# Autodesk Inventor assembly: gears
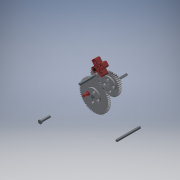
[picture p0: Inventor's stored thumbnail of the model, 180x180]
Saved by Autodesk Inventor 2019 (Build 230136000, 136)
## iProperties
Created: 2019-01-24
Part Number: gears
Document SubType Name: Assembly
Designer: Varga Daniel
Author: Varga Daniel
## Documents named in this file (8)
- C:\!_Dani\!_cloud\OneDrive\!_munka\Revolution\RevvyDemoKit\Structural parts\Demo parts\Gears\gears.iam
- C:\!_Dani\!_cloud\OneDrive\!_munka\Revolution\RevvyDemoKit\Structural parts\Connetor Pins\cp1x1.ipt
- C:\!_Dani\!_cloud\OneDrive\!_munka\Revolution\RevvyDemoKit\Structural parts\Axle Connectors\Axle connector 3x3 cross.ipt
- C:\!_Dani\!_cloud\OneDrive\!_munka\Revolution\RevvyDemoKit\Structural parts\Demo parts\Gears\gear40.iam
- C:\!_Dani\!_cloud\OneDrive\!_munka\Revolution\RevvyDemoKit\Structural parts\Axles\Axle 2.ipt
- C:\!_Dani\!_cloud\OneDrive\!_munka\Revolution\RevvyDemoKit\Structural parts\Demo parts\Gears\gear60.iam
- C:\!_Dani\!_cloud\OneDrive\!_munka\Revolution\RevvyDemoKit\Structural parts\Axles\Axle 5s.ipt
- C:\!_Dani\!_cloud\OneDrive\!_munka\Revolution\RevvyDemoKit\Structural parts\Demo parts\Gears\gear20.iam
## Components (12 placed, 7 different names)
1. cp1x1:1 — Mate:3, Mate:4
2. gear40:1 [sub-assembly] — Mate:12, Mate:13, Flush:1, Mate:16, Mate:18, Mate:19, Mate:20
3. Axle connector 3x3 cross:2 — Mate:3, Mate:4
4. gear60:1 [sub-assembly] — Mate:8, Mate:9, Mate:10, Mate:11, Flush:2, Mate:17, Angle:1, Mate:18
5. Axle 2:3
6. Axle 2:4 — Mate:8, Mate:9, Angle:1
7. cp1x1:2 — Mate:10, Mate:11
8. Axle 5s:1
9. Axle 5s:2 — Mate:12, Mate:13
10. gear20:1 [sub-assembly] — Mate:14, Mate:15, Flush:1, Mate:16, Flush:2, Mate:17
11. Axle 5s:3 — Mate:14, Mate:15
12. gear20:2 [sub-assembly] — Mate:19, Mate:20
## Relationships (18: Mate 15, Flush 2, Angle 1)
- Mate:3: cp1x1:1 ↔ Axle connector 3x3 cross:2
- Mate:4: cp1x1:1 ↔ Axle connector 3x3 cross:2
- Mate:8: gear60:1 ↔ Axle 2:4
- Mate:9: gear60:1 ↔ Axle 2:4
- Mate:10: gear60:1 ↔ cp1x1:2
- Mate:11: gear60:1 ↔ cp1x1:2
- Mate:12: gear40:1 ↔ Axle 5s:2
- Mate:13: gear40:1 ↔ Axle 5s:2
- Mate:14: gear20:1 ↔ Axle 5s:3
- Mate:15: gear20:1 ↔ Axle 5s:3
- Flush:1: gear40:1 ↔ gear20:1
- Mate:16 (30 mm): gear40:1 ↔ gear20:1
- Flush:2: gear60:1 ↔ gear20:1
- Mate:17 (40 mm): gear60:1 ↔ gear20:1
- Angle:1 (0 deg): gear60:1 ↔ Axle 2:4
- Mate:18 (50 mm): gear40:1 ↔ gear60:1
- Mate:19: gear40:1 ↔ gear20:2
- Mate:20: gear40:1 ↔ gear20:2
